# Autodesk Inventor assembly: vane_mirror_pattern
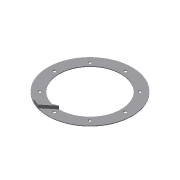
[picture p0: Inventor's stored thumbnail of the model, 180x180]
Saved by Autodesk Inventor 2022 (Build 260148000, 148)
## iProperties
Created: 2006-08-01
Part Number: vane_mirror_pattern
Document SubType Name: Assembly
Designer: jmacmillan
Author: jmacmillan
## Documents named in this file (3)
- C:\Autodesk Inventor 2022 Advanced Assembly Modeling Practice Files\Mirror and Pattern\vane_mirror_pattern.iam
- C:\Autodesk Inventor 2022 Advanced Assembly Modeling Practice Files\Mirror and Pattern\Vane_Plate.ipt
- C:\Autodesk Inventor 2022 Advanced Assembly Modeling Practice Files\Mirror and Pattern\Vane_blade.ipt
## Components (2 placed, 2 different names)
1. Vane_Plate:1 — Insert:1
2. Vane_blade:1 — Insert:1, Angle:1
## Relationships (2: Insert 1, Angle 1)
- Insert:1: Vane_Plate:1 ↔ Vane_blade:1
- Angle:1 (0 deg): Vane_blade:1
